# Autodesk Inventor assembly: ASY MSC 03 монтаж
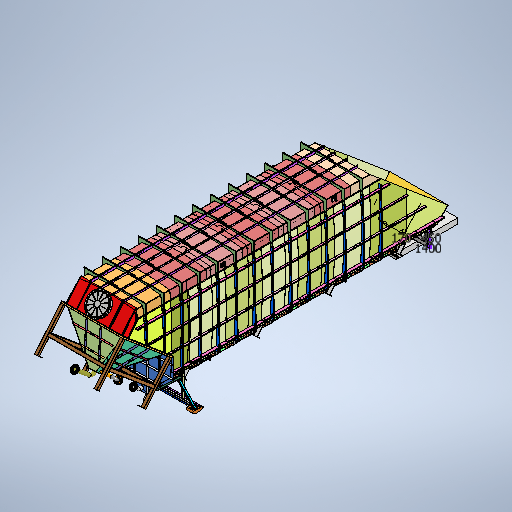
[picture p0: Inventor's stored thumbnail of the model, 512x512]
Saved by Autodesk Inventor 2025.1 (Build 291241020, 241B)
## iProperties
Created: 2024-11-20
Part Number: ASY MSC 03 монтаж
Document SubType Name: Assembly
Designer: user
Author: user
## Documents named in this file (5)
- C:\Users\user\YandexDisk-badmisterfox\домашниий пк\Inventor\Manturovo\Manturovo_Se-clar\ASY MSC 03 монтаж.iam
- C:\Users\user\YandexDisk-badmisterfox\домашниий пк\Inventor\Manturovo\Manturovo_Se-clar\ASY MSC 002 отстойник осветлитель.iam
- C:\Users\user\YandexDisk-badmisterfox\домашниий пк\Inventor\Manturovo\Manturovo_Se-clar\3d party\floor.ipt
- C:\Users\user\YandexDisk-badmisterfox\домашниий пк\Inventor\Manturovo\Manturovo_Se-clar\ASY MSC 2000 carriage.iam
- C:\Users\user\YandexDisk-badmisterfox\домашниий пк\Inventor\Manturovo\Manturovo_Se-clar\ASY MSC 3000 carriage nose.iam
## Components (4 placed, 4 different names)
1. ASY MSC 002 отстойник осветлитель:1 [sub-assembly] — Mate:1, Mate:2, Mate:5
2. floor:1 — Flush:1
3. ASY MSC 2000 carriage:1 [sub-assembly] — Flush:2, Mate:5
4. ASY MSC 3000 carriage nose:1 [sub-assembly] — Flush:5, Mate:4
## Relationships (8: Mate 5, Flush 3)
- Mate:1 (50 mm): ASY MSC 002 отстойник осветлитель:1
- Flush:1: floor:1
- Mate:2: ASY MSC 002 отстойник осветлитель:1
- [Mate]: floor:1 ↔ ASY MSC 2000 carriage:1
- Flush:2: ASY MSC 2000 carriage:1
- Flush:5: ASY MSC 3000 carriage nose:1
- Mate:4: ASY MSC 3000 carriage nose:1
- Mate:5: ASY MSC 002 отстойник осветлитель:1 ↔ ASY MSC 2000 carriage:1
